# Autodesk Inventor assembly: Ensamble Controlador
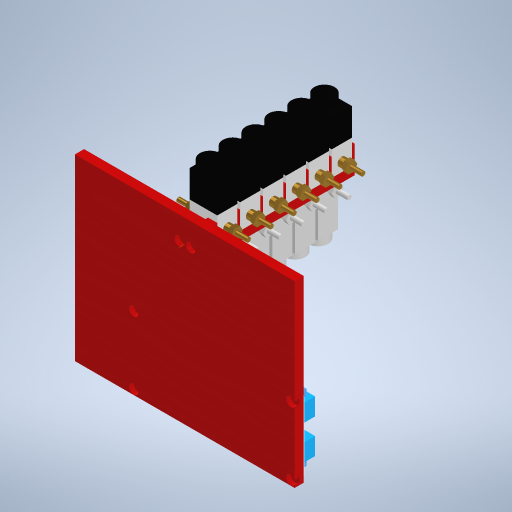
[picture p0: Inventor's stored thumbnail of the model, 512x512]
Saved by Autodesk Inventor 2024.2 (Build 282272000, 272)
## iProperties
Created: 2024-05-09
Part Number: Ensamble Controlador
Document SubType Name: Assembly
Designer: jp.reyesf
Author: jp.reyesf
## Documents named in this file (3)
- C:\Users\jp.reyesf\Desktop\SoftRobotics\Proyecto\CAD\Control\Ensamble Controlador.iam
- C:\Users\jp.reyesf\Desktop\SoftRobotics\Proyecto\CAD\Control\16 RELAY MODULE LOW LEVEL TRIGGER.ipt
- C:\Users\jp.reyesf\Desktop\SoftRobotics\Proyecto\CAD\Control\Montaje Valvulas.ipt
## Components (2 placed, 2 different names)
1. 16 RELAY MODULE LOW LEVEL TRIGGER:1 — Mate:1, Mate:2, Mate:3
2. Montaje Valvulas:1 — Mate:1, Mate:2, Mate:3
## Relationships (3: Mate 3)
- Mate:1: 16 RELAY MODULE LOW LEVEL TRIGGER:1 ↔ Montaje Valvulas:1
- Mate:2: 16 RELAY MODULE LOW LEVEL TRIGGER:1 ↔ Montaje Valvulas:1
- Mate:3: 16 RELAY MODULE LOW LEVEL TRIGGER:1 ↔ Montaje Valvulas:1
